# Autodesk Inventor assembly: Robot
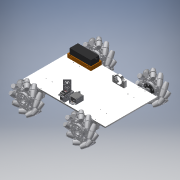
[picture p0: Inventor's stored thumbnail of the model, 180x180]
Saved by Autodesk Inventor 2017 (Build 210142000, 142)
## iProperties
Created: 2017-09-30
Part Number: Robot
Document SubType Name: Assembly
Designer: User
Author: User
## Documents named in this file (7)
- C:\Robotics\CAD\2017-18_CAD\Robot.iam
- C:\Robotics\CAD\2017-18_CAD\PlateFrame1.ipt
- C:\Robotics\CAD\2017-18_CAD\DirectDriveMotorSubAsembly.iam
- C:\Robotics\CAD\2017-18_CAD\batery.ipt
- C:\Robotics\CAD\2017-18_CAD\batteryholder.ipt
- C:\Robotics\CAD\2017-18_CAD\JewlArm.iam
- C:\Robotics\CAD\COTSParts\Tetrix\tetrix-motor-mounts-1.snapshot.1\Tetrex 2pc motor mount.ipt
## Components (9 placed, 6 different names)
1. PlateFrame1:1 — Mate:1, Mate:2, Mate:3, Mate:4, Mate:6, Mate:7, Mate:8, Mate:11, Mate:12, Mate:14, Mate:15, Mate:16, Mate:17, Mate:26, Mate:39, Flush:14, Flush:15, Mate:40, Flush:18, Flush:19, Flush:20, Flush:21
2. DirectDriveMotorSubAsembly:1 [sub-assembly] — Mate:1, Mate:2, Mate:3
3. DirectDriveMotorSubAsembly:2 [sub-assembly] — Mate:14, Mate:15, Mate:16
4. DirectDriveMotorSubAsembly:3 [sub-assembly] — Mate:11, Mate:12, Mate:17
5. DirectDriveMotorSubAsembly:4 [sub-assembly] — Mate:4, Mate:6, Mate:7, Mate:8
6. batery:1 — Mate:23, Mate:41, Mate:42
7. batteryholder:1 — Mate:23, Mate:26, Flush:18, Flush:19, Mate:41, Mate:42
8. JewlArm:1 [sub-assembly] — Mate:39, Flush:14, Flush:15
9. Tetrex 2pc motor mount:1 — Mate:40, Flush:20, Flush:21
## Relationships (25: Mate 19, Flush 6)
- Mate:1: PlateFrame1:1 ↔ DirectDriveMotorSubAsembly:1
- Mate:2: PlateFrame1:1 ↔ DirectDriveMotorSubAsembly:1
- Mate:3: PlateFrame1:1 ↔ DirectDriveMotorSubAsembly:1
- Mate:4: PlateFrame1:1 ↔ DirectDriveMotorSubAsembly:4
- Mate:6: PlateFrame1:1 ↔ DirectDriveMotorSubAsembly:4
- Mate:7: PlateFrame1:1 ↔ DirectDriveMotorSubAsembly:4
- Mate:8: PlateFrame1:1 ↔ DirectDriveMotorSubAsembly:4
- Mate:11: PlateFrame1:1 ↔ DirectDriveMotorSubAsembly:3
- Mate:12: PlateFrame1:1 ↔ DirectDriveMotorSubAsembly:3
- Mate:14: PlateFrame1:1 ↔ DirectDriveMotorSubAsembly:2
- Mate:15: PlateFrame1:1 ↔ DirectDriveMotorSubAsembly:2
- Mate:16: PlateFrame1:1 ↔ DirectDriveMotorSubAsembly:2
- Mate:17: PlateFrame1:1 ↔ DirectDriveMotorSubAsembly:3
- Mate:23: batery:1 ↔ batteryholder:1
- Mate:26: PlateFrame1:1 ↔ batteryholder:1
- Mate:39 (12.7 mm): PlateFrame1:1 ↔ JewlArm:1
- Flush:14: PlateFrame1:1 ↔ JewlArm:1
- Flush:15 (207.5307 mm): PlateFrame1:1 ↔ JewlArm:1
- Mate:40: PlateFrame1:1 ↔ Tetrex 2pc motor mount:1
- Flush:18 (1.5875 mm): PlateFrame1:1 ↔ batteryholder:1
- Flush:19 (19.05 mm): PlateFrame1:1 ↔ batteryholder:1
- Mate:41: batery:1 ↔ batteryholder:1
- Mate:42: batery:1 ↔ batteryholder:1
- Flush:20 (127 mm): PlateFrame1:1 ↔ Tetrex 2pc motor mount:1
- Flush:21 (-38.1 mm): PlateFrame1:1 ↔ Tetrex 2pc motor mount:1
